# Autodesk Inventor assembly: Creat iAssembly
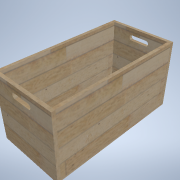
[picture p0: Inventor's stored thumbnail of the model, 180x180]
Saved by Autodesk Inventor 2021 (Build 250183000, 183)
## iProperties
RuleStatus: InUse
Created: 2020-08-22
Part Number: Creat iAssembly
Document SubType Name: Assembly
Designer: Oghenemarho Orukele
AfterDocOpen0: OnStart
Author: Oghenemarho Orukele
## Documents named in this file (6)
- C:\Users\Oghenemarho\Documents\Mars Manufacturing\iLogic Designs\Wooden Creat\Creat iAssembly.iam
- C:\Users\Oghenemarho\Documents\Mars Manufacturing\iLogic Designs\Wooden Creat\Creat Buttom-01.ipt
- C:\Users\Oghenemarho\Documents\Mars Manufacturing\iLogic Designs\Wooden Creat\Creat Front-01.ipt
- C:\Users\Oghenemarho\Documents\Mars Manufacturing\iLogic Designs\Wooden Creat\Creat Front-02.ipt
- C:\Users\Oghenemarho\Documents\Mars Manufacturing\iLogic Designs\Wooden Creat\Creat Side-01.ipt
- C:\Users\Oghenemarho\Documents\Mars Manufacturing\iLogic Designs\Wooden Creat\Creat Side-02.ipt
## Components (5 placed, 5 different names)
1. Creat Bottom-01:1 — Mate:8, Mate:9, Mate:10
2. Creat Front-01:1 — Mate:1, Mate:2, Mate:8
3. Creat Front-02:1 — Mate:6, Mate:7, Mate:10, Mate:11, Mate:12, Mate:13
4. Creat Side-01:1 — Mate:1, Mate:2, Mate:6, Mate:7, Mate:9
5. Creat Side-02:1 — Mate:11, Mate:12, Mate:13
## Relationships (10: Mate 10)
- Mate:1: Creat Front-01:1 ↔ Creat Side-01:1
- Mate:2: Creat Front-01:1 ↔ Creat Side-01:1
- Mate:6: Creat Front-02:1 ↔ Creat Side-01:1
- Mate:7: Creat Front-02:1 ↔ Creat Side-01:1
- Mate:8: Creat Bottom-01:1 ↔ Creat Front-01:1
- Mate:9: Creat Bottom-01:1 ↔ Creat Side-01:1
- Mate:10: Creat Bottom-01:1 ↔ Creat Front-02:1
- Mate:11: Creat Front-02:1 ↔ Creat Side-02:1
- Mate:12: Creat Front-02:1 ↔ Creat Side-02:1
- Mate:13: Creat Front-02:1 ↔ Creat Side-02:1
## Named parameters: Length = 500 mm, Width = 250 mm, Height = 250 mm, Thickness = 12.7 mm
